# Autodesk Inventor assembly: Magnet Panel for 4040 - Assembly
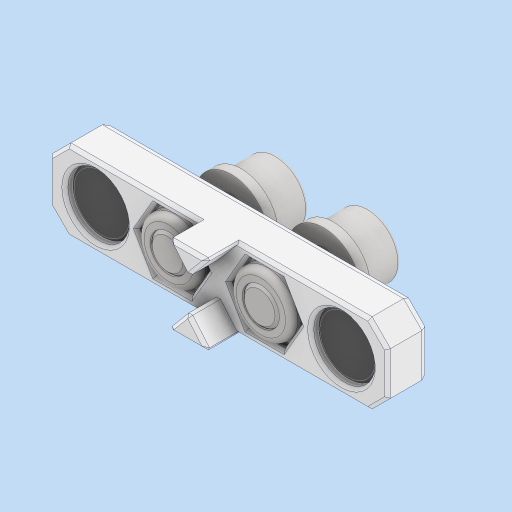
[picture p0: Inventor's stored thumbnail of the model, 512x512]
Saved by Autodesk Inventor 2023.2 (Build 272271000, 271)
## iProperties
Created: 2023-11-30
Part Number: Magnet Panel for 4040 - Assembly
Document SubType Name: Assembly
Designer: Nils Bade
Author: Nils Bade
## Documents named in this file (7)
- C:\Users\nilsb\Documents\Inventor\Projektarbeit-Bade\Enclosure\Magnet Panel for 4040 - Assembly.iam
- C:\Users\nilsb\Documents\Inventor\Projektarbeit-Bade\Enclosure\Magnet Panel for 4040.ipt
- C:\Users\nilsb\Documents\Inventor\Projektarbeit-Bade\Enclosure\Magnet-RatrigEnclosure.ipt
- C:\Users\nilsb\Documents\Inventor\Projektarbeit-Bade\RatRig_Standards\Hex Locking Nut - M6 v2.ipt
- C:\Users\nilsb\Documents\Inventor\Projektarbeit-Bade\Schrauben\Cap Head Screw M6x12 v2.ipt
- C:\Users\nilsb\Documents\Inventor\Projektarbeit-Bade\Schrauben\Washer Simple M6 v2.ipt
- Washer Simple M6 1,6mm.ipt
## Components (9 placed, 5 different names)
1. Magnet Panel for 4040:1 — Passend:1, Passend:2, Passend:3, Passend:4, Passend:5, Passend:6, Winkel:1, Winkel:2, Passend:7, Passend:8
2. Magnet-RatrigEnclosure:1 — Passend:1, Passend:3
3. Magnet-RatrigEnclosure:2 — Passend:2, Passend:4
4. Cap Head Screw M6x12 v2:1 — Passend:13, Passend:15
5. Cap Head Screw M6x12 v2:2 — Passend:14, Passend:16
6. Hex Locking Nut - M6 v2:1 — Passend:5, Winkel:1, Passend:7
7. Hex Locking Nut - M6 v2:2 — Passend:6, Winkel:2, Passend:8
8. Washer Simple M6 1,6mm:1 — Passend:13, Passend:15
9. Washer Simple M6 1,6mm:2 — Passend:14, Passend:16
## Relationships (18: Mate 16, Angle 2)
- Passend:1 [Mate]: Magnet Panel for 4040:1 ↔ Magnet-RatrigEnclosure:1
- Passend:2 [Mate]: Magnet Panel for 4040:1 ↔ Magnet-RatrigEnclosure:2
- Passend:3 [Mate]: Magnet Panel for 4040:1 ↔ Magnet-RatrigEnclosure:1
- Passend:4 [Mate]: Magnet Panel for 4040:1 ↔ Magnet-RatrigEnclosure:2
- Passend:5 [Mate]: Magnet Panel for 4040:1 ↔ Hex Locking Nut - M6 v2:1
- Passend:6 [Mate]: Magnet Panel for 4040:1 ↔ Hex Locking Nut - M6 v2:2
- Winkel:1 [Angle] (0 deg): Magnet Panel for 4040:1 ↔ Hex Locking Nut - M6 v2:1
- Winkel:2 [Angle] (0 deg): Magnet Panel for 4040:1 ↔ Hex Locking Nut - M6 v2:2
- Passend:7 [Mate]: Magnet Panel for 4040:1 ↔ Hex Locking Nut - M6 v2:1
- Passend:8 [Mate]: Magnet Panel for 4040:1 ↔ Hex Locking Nut - M6 v2:2
- [Mate]: Magnet Panel for 4040:1 ↔ Cap Head Screw M6x12 v2:2
- [Mate] (4.6 mm): Magnet Panel for 4040:1 ↔ Cap Head Screw M6x12 v2:2
- [Mate]: Magnet Panel for 4040:1 ↔ Cap Head Screw M6x12 v2:1
- [Mate] (4.6 mm): Magnet Panel for 4040:1 ↔ Cap Head Screw M6x12 v2:1
- Passend:13 [Mate]: Cap Head Screw M6x12 v2:1 ↔ Washer Simple M6 1,6mm:1
- Passend:14 [Mate]: Cap Head Screw M6x12 v2:2 ↔ Washer Simple M6 1,6mm:2
- Passend:15 [Mate]: Cap Head Screw M6x12 v2:1 ↔ Washer Simple M6 1,6mm:1
- Passend:16 [Mate]: Cap Head Screw M6x12 v2:2 ↔ Washer Simple M6 1,6mm:2
